# Autodesk Inventor assembly: サイクロイド減速機
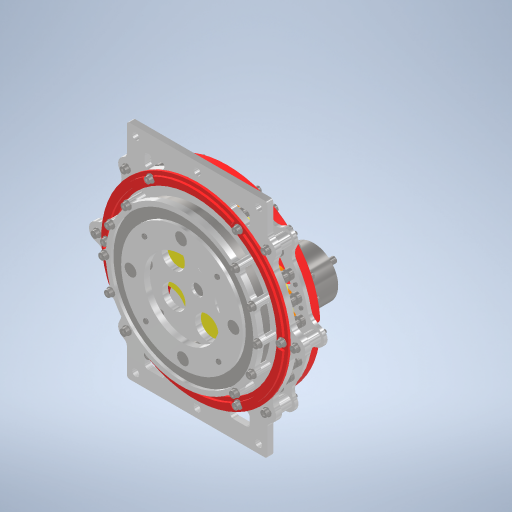
[picture p0: Inventor's stored thumbnail of the model, 512x512]
Saved by Autodesk Inventor 2024 (Build 280153000, 153)
## iProperties
Created: 2023-05-29
Part Number: サイクロイド減速機
Document SubType Name: Assembly
Designer: yuta2
Mass: 2083.84 g
Surface Area: 3326.87 cm^2
Volume: 587.86 cm^3
Density: 3.54478 g/cm^3
Author: yuta2
## Documents named in this file (27)
- C:\Users\yuta2\Documents\Inventor\CycloidDrive\サイクロイド減速機_大型\サイクロイド減速機.iam
- C:\Users\yuta2\Documents\Inventor\CycloidDrive\サイクロイド減速機_大型\サイクロイド減速機パラメータ.ipt
- C:\Users\yuta2\Documents\Inventor\CycloidDrive\サイクロイド減速機_大型\サイクロイドギア.ipt
- C:\Users\yuta2\Documents\Inventor\CycloidDrive\サイクロイド減速機_大型\ベース板_出力側.ipt
- C:\Users\yuta2\Documents\Inventor\CycloidDrive\サイクロイド減速機_大型\偏心軸ユニット.iam
- C:\Users\yuta2\Documents\Inventor\CycloidDrive\サイクロイド減速機_大型\出力板ユニット.iam
- C:\Users\yuta2\Documents\Inventor\CycloidDrive\サイクロイド減速機_大型\入力軸.ipt
- C:\Users\yuta2\Documents\Inventor\CycloidDrive\サイクロイド減速機_大型\出力ベアリング抑え.ipt
- C:\Users\yuta2\Documents\Inventor\CycloidDrive\サイクロイド減速機_大型\スペーサCL-309E.ipt
- C:\Users\yuta2\Documents\Inventor\CycloidDrive\サイクロイド減速機_大型\サイクロイド減速機\デザイン アクセラレータ\ボルト締結1.iam
- C:\Users\yuta2\Documents\Inventor\CycloidDrive\サイクロイド減速機_大型\外周ピンユニット.iam
- C:\Users\yuta2\Documents\Inventor\CycloidDrive\サイクロイド減速機_大型\ベース板入力側.ipt
- C:\Users\yuta2\Documents\Inventor\CycloidDrive\ベアリング\SMF148ZZ.ipt
- C:\Users\yuta2\Documents\Inventor\CycloidDrive\ベアリング\676ZZ.ipt
- C:\Users\yuta2\Documents\Inventor\CycloidDrive\サイクロイド減速機_大型\RZ735.ipt
- C:\Users\yuta2\Documents\Inventor\CycloidDrive\サイクロイド減速機_大型\サイクロイド減速機\デザイン アクセラレータ\平歯車1.iam
- C:\Users\yuta2\Documents\Inventor\CycloidDrive\サイクロイド減速機_大型\サイクロイド減速機\デザイン アクセラレータ\平歯車2.iam
- C:\Users\yuta2\Documents\Inventor\CycloidDrive\サイクロイド減速機_大型\モーターマウント板.ipt
- C:\Users\yuta2\Documents\Inventor\CycloidDrive\サイクロイド減速機_大型\モーターマウント板固定部品.ipt
- C:\Users\yuta2\Documents\Inventor\CycloidDrive\サイクロイド減速機_大型\モーターマウント板固定部品2.ipt
- C:\Users\yuta2\Documents\Inventor\CycloidDrive\共通部品\インサートナットM4.ipt
- C:\Users\yuta2\Documents\Inventor\CycloidDrive\サイクロイド減速機_大型\サイクロイド減速機\デザイン アクセラレータ\ボルト締結2.iam
- C:\Users\yuta2\Documents\Inventor\CycloidDrive\サイクロイド減速機_大型\サイクロイド減速機\デザイン アクセラレータ\ボルト締結3.iam
- C:\Users\yuta2\Documents\Inventor\CycloidDrive\サイクロイド減速機_大型\外周ピン抑え.ipt
- C:\Users\yuta2\Documents\Inventor\CycloidDrive\サイクロイド減速機_大型\サイクロイド減速機\デザイン アクセラレータ\ボルト締結4.iam
- C:\Users\yuta2\Documents\Inventor\CycloidDrive\サイクロイド減速機_大型\ベース板連結棒.ipt
- C:\Users\yuta2\Documents\Inventor\CycloidDrive\サイクロイド減速機_大型\サイクロイド減速機\デザイン アクセラレータ\ボルト締結5.iam
## Components (91 placed, 21 different names)
1. サイクロイド減速機パラメータ:1
2. サイクロイドギア:1 — 回転:1
3. ベース板_出力側:1 — 回転:3, 回転:8, 回転:9, 回転:25, 回転:26, メイト:11, メイト:12
4. 偏心軸ユニット:1 [sub-assembly] — 回転:1, 回転:2, 回転:5, 回転:10
5. サイクロイドギア:2 — 回転:2
6. 出力板ユニット:1 [sub-assembly] — 回転:3, 回転:4, 回転:5, 回転:6
7. 入力軸:1 — 回転:4, 回転:12
8. 出力ベアリング抑え:1 — 回転:6, 回転:7, メイト:1, メイト:2
9. ボルト締結:1 [sub-assembly] — メイト:1, メイト:2
10. ベース板入力側:1 — 円柱状:1, 回転:10, 回転:11, 回転:13, 回転:17, 回転:24, メイト:6, 回転:27
11. SMF148ZZ:1 — 回転:11
12. 676ZZ:1 — 回転:12, 円柱状:2
13. RZ735:1 — 回転:14, 回転:15, 回転:16
14. 平歯車:1 [sub-assembly] — 回転:13
15. 平歯車:2 [sub-assembly] — 回転:14
16. モーターマウント板:1 — 回転:15, 回転:16, 円柱状:2, 回転:18, 回転:19, 回転:20, 回転:21, メイト:9, メイト:10
17. モーターマウント板固定部品:1 — 回転:17, 回転:18, 回転:19, 回転:22, 回転:24, メイト:5
18. モーターマウント板固定部品2:1 — 回転:20, 回転:21, 回転:23
19. ボルト締結:2 [sub-assembly] — メイト:9, メイト:10
20. ボルト締結:3 [sub-assembly] — メイト:5, メイト:6
21. 外周ピン抑え:1 — 回転:25, 回転:26, メイト:7, メイト:8
22. 外周ピンユニット:1 [sub-assembly] — 回転:9, 円柱状:1
23. 外周ピンユニット:2 [sub-assembly]
24. 外周ピンユニット:3 [sub-assembly]
25. 外周ピンユニット:4 [sub-assembly]
26. 外周ピンユニット:5 [sub-assembly]
27. 外周ピンユニット:6 [sub-assembly]
28. 外周ピンユニット:7 [sub-assembly]
29. 外周ピンユニット:8 [sub-assembly]
30. 外周ピンユニット:9 [sub-assembly]
31. 外周ピンユニット:10 [sub-assembly]
32. 外周ピンユニット:11 [sub-assembly]
33. 外周ピンユニット:12 [sub-assembly]
34. 外周ピンユニット:13 [sub-assembly]
35. 外周ピンユニット:14 [sub-assembly]
36. 外周ピンユニット:15 [sub-assembly]
37. 外周ピンユニット:16 [sub-assembly]
38. 外周ピンユニット:17 [sub-assembly]
39. 外周ピンユニット:18 [sub-assembly]
40. 外周ピンユニット:19 [sub-assembly]
41. 外周ピンユニット:20 [sub-assembly]
42. 外周ピンユニット:21 [sub-assembly]
43. 外周ピンユニット:22 [sub-assembly]
44. 外周ピンユニット:23 [sub-assembly]
45. 外周ピンユニット:24 [sub-assembly]
46. 外周ピンユニット:25 [sub-assembly]
47. 外周ピンユニット:26 [sub-assembly]
48. 外周ピンユニット:27 [sub-assembly]
49. 外周ピンユニット:28 [sub-assembly]
50. 外周ピンユニット:29 [sub-assembly]
51. 外周ピンユニット:30 [sub-assembly]
52. インサートナットM4:1 — 回転:22
53. インサートナットM4:3
54. インサートナットM4:4
55. インサートナットM4:5
56. インサートナットM4:6
57. インサートナットM4:7
58. インサートナットM4:2 — 回転:23
59. インサートナットM4:8
60. インサートナットM4:9
61. インサートナットM4:10
62. インサートナットM4:11
63. インサートナットM4:12
64. ボルト締結:4 [sub-assembly] — メイト:7, メイト:8
65. ボルト締結:5 [sub-assembly]
66. ボルト締結:6 [sub-assembly]
67. ボルト締結:7 [sub-assembly]
68. ボルト締結:8 [sub-assembly]
69. ボルト締結:9 [sub-assembly]
70. スペーサCL-309E:1 — 回転:7, 回転:8
71. スペーサCL-309E:2
72. スペーサCL-309E:3
73. スペーサCL-309E:4
74. スペーサCL-309E:5
75. スペーサCL-309E:6
76. スペーサCL-309E:7
77. スペーサCL-309E:8
78. スペーサCL-309E:9
79. スペーサCL-309E:10
80. ベース板連結棒:1 — 回転:27
81. ベース板連結棒:2
82. ベース板連結棒:3
83. ベース板連結棒:4
84. ベース板連結棒:5
85. ベース板連結棒:6
86. ボルト締結:10 [sub-assembly] — メイト:11, メイト:12
87. ボルト締結:11 [sub-assembly]
88. ボルト締結:12 [sub-assembly]
89. ボルト締結:13 [sub-assembly]
90. ボルト締結:14 [sub-assembly]
91. ボルト締結:15 [sub-assembly]
## Component patterns: (2 elements), (30 elements, first: 外周ピンユニット:1), (6 elements, first: インサートナットM4:1), (6 elements, first: インサートナットM4:2), (6 elements, first: ボルト締結:4), (2 elements), (3 elements), (5 elements, first: スペーサCL-309E:1), コンポーネント パターン 1:2 (5 elements), (3 elements, first: ベース板連結棒:1), コンポーネント パターン 7:2 (3 elements), (2 elements, first: ボルト締結:10), コンポーネント パターン 9:2 (2 elements), コンポーネント パターン 9:3 (2 elements)
## Relationships (39: RevoluteJoint 27, Mate 10, CylindricalJoint 2)
- 回転:1 [RevoluteJoint]: サイクロイドギア:1 ↔ 偏心軸ユニット:1
- 回転:2 [RevoluteJoint]: 偏心軸ユニット:1 ↔ サイクロイドギア:2
- 回転:3 [RevoluteJoint]: ベース板_出力側:1 ↔ 出力板ユニット:1
- 回転:4 [RevoluteJoint]: 出力板ユニット:1 ↔ 入力軸:1
- 回転:5 [RevoluteJoint] (0.5 mm): 偏心軸ユニット:1 ↔ 出力板ユニット:1
- 回転:6 [RevoluteJoint]: 出力板ユニット:1 ↔ 出力ベアリング抑え:1
- 回転:7 [RevoluteJoint]: 出力ベアリング抑え:1 ↔ スペーサCL-309E:1
- 回転:8 [RevoluteJoint]: ベース板_出力側:1 ↔ スペーサCL-309E:1
- メイト:1 [Mate]: 出力ベアリング抑え:1 ↔ ボルト締結:1
- メイト:2 [Mate]: 出力ベアリング抑え:1 ↔ ボルト締結:1
- 回転:9 [RevoluteJoint]: ベース板_出力側:1 ↔ 外周ピンユニット:1
- 円柱状:1 [CylindricalJoint]: ベース板入力側:1 ↔ 外周ピンユニット:1
- 回転:10 [RevoluteJoint] (-0.5 mm): 偏心軸ユニット:1 ↔ ベース板入力側:1
- 回転:11 [RevoluteJoint]: ベース板入力側:1 ↔ SMF148ZZ:1
- 回転:12 [RevoluteJoint]: 入力軸:1 ↔ 676ZZ:1
- 回転:13 [RevoluteJoint] (1 mm): ベース板入力側:1 ↔ 平歯車:1
- 回転:14 [RevoluteJoint] (0.5 mm): RZ735:1 ↔ 平歯車:2
- 回転:15 [RevoluteJoint]: RZ735:1 ↔ モーターマウント板:1
- 回転:16 [RevoluteJoint]: RZ735:1 ↔ モーターマウント板:1
- 円柱状:2 [CylindricalJoint]: 676ZZ:1 ↔ モーターマウント板:1
- 回転:17 [RevoluteJoint]: ベース板入力側:1 ↔ モーターマウント板固定部品:1
- 回転:18 [RevoluteJoint]: モーターマウント板:1 ↔ モーターマウント板固定部品:1
- 回転:19 [RevoluteJoint]: モーターマウント板:1 ↔ モーターマウント板固定部品:1
- 回転:20 [RevoluteJoint]: モーターマウント板:1 ↔ モーターマウント板固定部品2:1
- 回転:21 [RevoluteJoint]: モーターマウント板:1 ↔ モーターマウント板固定部品2:1
- 回転:22 [RevoluteJoint]: モーターマウント板固定部品:1 ↔ インサートナットM4:1
- 回転:23 [RevoluteJoint]: モーターマウント板固定部品2:1 ↔ インサートナットM4:2
- 回転:24 [RevoluteJoint]: ベース板入力側:1 ↔ モーターマウント板固定部品:1
- メイト:5 [Mate]: モーターマウント板固定部品:1 ↔ ボルト締結:3
- メイト:6 [Mate]: ベース板入力側:1 ↔ ボルト締結:3
- 回転:25 [RevoluteJoint]: ベース板_出力側:1 ↔ 外周ピン抑え:1
- 回転:26 [RevoluteJoint]: ベース板_出力側:1 ↔ 外周ピン抑え:1
- メイト:7 [Mate]: 外周ピン抑え:1 ↔ ボルト締結:4
- メイト:8 [Mate]: 外周ピン抑え:1 ↔ ボルト締結:4
- メイト:9 [Mate]: モーターマウント板:1 ↔ ボルト締結:2
- メイト:10 [Mate]: モーターマウント板:1 ↔ ボルト締結:2
- 回転:27 [RevoluteJoint]: ベース板入力側:1 ↔ ベース板連結棒:1
- メイト:11 [Mate]: ベース板_出力側:1 ↔ ボルト締結:10
- メイト:12 [Mate]: ベース板_出力側:1 ↔ ボルト締結:10
## Named parameters: N_pin = 30, r = 2 mm, D = 150 mm, Dc = 4.83871 mm, D_pin = 8 mm
